# Autodesk Inventor assembly: ASY GBK 3120 central wall shield 2
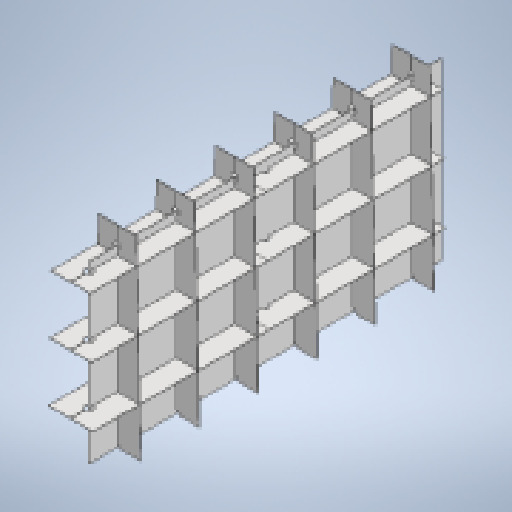
[picture p0: Inventor's stored thumbnail of the model, 512x512]
Saved by Autodesk Inventor 2026 (Build 300175000, 175)
## iProperties
Created: 2026-05-19
Part Number: ASY GBK 3120 central wall shield 2
Document SubType Name: Assembly
Designer: pokla
Mass: 174041 g
Surface Area: 113034 cm^2
Volume: 22170.8 cm^3
Density: 7.85 g/cm^3
Author: admin
## Documents named in this file (8)
- C:\Users\pokla\Documents\Inventor\GBK-Gubkinskiy\ASY GBK 3120 central wall shield 2.iam
- C:\Users\pokla\Documents\Inventor\GBK-Gubkinskiy\GBK 0101 main rib.ipt
- C:\Users\pokla\Documents\Inventor\GBK-Gubkinskiy\GBK 3122 shield 2.ipt
- C:\Users\pokla\Documents\Inventor\GBK-Gubkinskiy\GBK 3112 central main rib_CPY.ipt
- GBK 3112 central main rib_CPY.ipt
- C:\Users\pokla\Documents\Inventor\GBK-Gubkinskiy\GBK 3113 stringer 1.ipt
- C:\Users\pokla\Documents\Inventor\GBK-Gubkinskiy\GBK 3114 stringer 2.ipt
- C:\Users\pokla\Documents\Inventor\GBK-Gubkinskiy\GBK 3115 stringer 3.ipt
## Components (25 placed, 5 different names)
1. GBK 3113 stringer 1:1 — Жесткий:1, Жесткий:10
2. GBK 3122 shield 2:1 — Совмещение:1, Заподлицо:1, Совмещение:2, Заподлицо:3, Совмещение:5, Заподлицо:5, Заподлицо:2, Совмещение:4
3. GBK 3114 stringer 2:1 — Жесткий:2, Жесткий:11
4. GBK 3115 stringer 3:1 — Жесткий:3, Жесткий:12
5. GBK 3113 stringer 1:2 — Жесткий:6, Жесткий:7
6. GBK 3114 stringer 2:2 — Жесткий:5, Жесткий:8
7. GBK 3115 stringer 3:2 — Жесткий:6, Жесткий:9
8. GBK 3113 stringer 1:3 — Жесткий:7
9. GBK 3114 stringer 2:3 — Жесткий:8
10. GBK 3115 stringer 3:3 — Жесткий:9
11. GBK 3113 stringer 1:4 — Жесткий:10
12. GBK 3114 stringer 2:4 — Жесткий:11
13. GBK 3115 stringer 3:4 — Жесткий:12
14. GBK 3112 central main rib_CPY:2 — Заподлицо:3, Совмещение:5, Заподлицо:5, Заподлицо:4, Жесткий:3, Жесткий:2, Жесткий:1
15. GBK 3112 central main rib_CPY:3
16. GBK 3112 central main rib_CPY:4
17. GBK 3112 central main rib_CPY:10
18. GBK 3112 central main rib_CPY:11
19. GBK 3112 central main rib_CPY:12
20. GBK 3112 central main rib_CPY:1 — Заподлицо:2, Совмещение:4, Заподлицо:4, Жесткий:6, Жесткий:5, Жесткий:6
21. GBK 3112 central main rib_CPY:5
22. GBK 3112 central main rib_CPY:6
23. GBK 3112 central main rib_CPY:7
24. GBK 3112 central main rib_CPY:8
25. GBK 3112 central main rib_CPY:9
## Component patterns: (6 elements, first: GBK 3112 central main rib_CPY:2), (6 elements, first: GBK 3112 central main rib_CPY:1)
## Relationships (21: WeldJoint 12, Flush 5, Mate 4)
- Совмещение:1 [Mate]: GBK 3122 shield 2:1
- Заподлицо:1 [Flush]: GBK 3122 shield 2:1
- Совмещение:2 [Mate]: GBK 3122 shield 2:1
- Заподлицо:3 [Flush]: GBK 3122 shield 2:1 ↔ GBK 3112 central main rib_CPY:2
- Совмещение:5 [Mate]: GBK 3122 shield 2:1 ↔ GBK 3112 central main rib_CPY:2
- Заподлицо:5 [Flush] (254 mm): GBK 3122 shield 2:1 ↔ GBK 3112 central main rib_CPY:2
- Заподлицо:2 [Flush]: GBK 3122 shield 2:1 ↔ GBK 3112 central main rib_CPY:1
- Совмещение:4 [Mate]: GBK 3122 shield 2:1 ↔ GBK 3112 central main rib_CPY:1
- Заподлицо:4 [Flush]: GBK 3112 central main rib_CPY:2 ↔ GBK 3112 central main rib_CPY:1
- Жесткий:3 [WeldJoint] (4 mm): GBK 3115 stringer 3:1 ↔ GBK 3112 central main rib_CPY:2
- Жесткий:2 [WeldJoint] (4 mm): GBK 3114 stringer 2:1 ↔ GBK 3112 central main rib_CPY:2
- Жесткий:1 [WeldJoint] (4 mm): GBK 3113 stringer 1:1 ↔ GBK 3112 central main rib_CPY:2
- Жесткий:6 [WeldJoint] (4 mm): GBK 3113 stringer 1:2 ↔ GBK 3112 central main rib_CPY:1
- Жесткий:5 [WeldJoint] (4 mm): GBK 3114 stringer 2:2 ↔ GBK 3112 central main rib_CPY:1
- Жесткий:6 [WeldJoint] (4 mm): GBK 3115 stringer 3:2 ↔ GBK 3112 central main rib_CPY:1
- Жесткий:7 [WeldJoint]: GBK 3113 stringer 1:2 ↔ GBK 3113 stringer 1:3
- Жесткий:8 [WeldJoint]: GBK 3114 stringer 2:2 ↔ GBK 3114 stringer 2:3
- Жесткий:9 [WeldJoint]: GBK 3115 stringer 3:2 ↔ GBK 3115 stringer 3:3
- Жесткий:10 [WeldJoint]: GBK 3113 stringer 1:1 ↔ GBK 3113 stringer 1:4
- Жесткий:11 [WeldJoint]: GBK 3114 stringer 2:1 ↔ GBK 3114 stringer 2:4
- Жесткий:12 [WeldJoint]: GBK 3115 stringer 3:1 ↔ GBK 3115 stringer 3:4
## Named parameters: основание_длина_нижнего = 196 mm, основание_длина_верхнего = 96 mm, стрингер_глубина_1 = 186.70056 mm, стрингер_глубина_2 = 175.35977 mm, стрингер_глубина_3 = 164.01899 mm, стрингер_глубина_4 = 152.6782 mm, стрингер_глубина_5 = 141.33742 mm, стрингер_глубина_6 = 129.99663 mm, стрингер_глубина_7 = 118.65585 mm, стрингер_глубина_8 = 107.31507 mm, Лист_ширина = 1480 mm, ребро_усилителей = 60 mm, паз_под_стрингер_глубина = 70 mm, паз_под_стрингер_толщина = 5 mm, отступ_от_пола_до_первого_стрингера = 410 mm, шаг_стрингеров = 500 mm, радиус_выреза_под_сварку = 30 mm, нахлест_шпангоутов_1_2 = 150 mm, нахлест_шпангоутов_2_3 = 120 mm, Стрингер_длина = 1490 mm, Лист_длина = 2980 mm, Шаг_шпангоутов = 496.66667 mm
